# Autodesk Inventor assembly: mg996r 3mm center frame
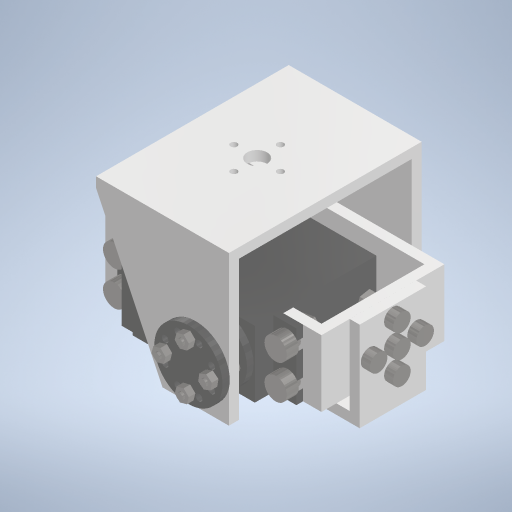
[picture p0: Inventor's stored thumbnail of the model, 512x512]
Saved by Autodesk Inventor 2023 (Build 270158000, 158)
## iProperties
Created: 2022-06-29
Part Number: mg996r 3mm center frame
Document SubType Name: Assembly
Designer: isamu
Author: isamu
## iProperties of the stored document servo frame mg996 centered.ipt
Created: 2022-06-29
Part Number: Pocket036
Material: Generic
Description: FreeCAD Model
Document SubType Name: Modeling
Designer: isamu
Authority: Unknown
Density: 1 g/cm^3
Appearance: Default
Title: Open CASCADE Shape Model
Author: Author
Sending System: FreeCAD
Preprocessor: Open CASCADE STEP processor 7.5
## Documents named in this file (7)
- **D:\personal_projects\robot\inventor\mg996r 3mm center frame.iam*LocalDocs*xAaaaawdaAaaaaaaaAaaaajx33d*servo frame mg996 centered.ipt
- D:\personal_projects\robot\inventor\mg996r 3mm center frame.iam
- D:\personal_projects\robot\inventor\base mg996r 3mm with bottom.iam
- D:\personal_projects\robot\exports\frames\m4 nuts.ipt
- D:\personal_projects\robot\exports\frames\m2x8.ipt
- D:\personal_projects\robot\exports\frames\m2 nuts.ipt
- D:\personal_projects\robot\exports\frames\servo frame mg996 centered.step
## Components (11 placed, 5 different names)
1. base mg996r 3mm with bottom:1 [sub-assembly] — Insert:6, Insert:7, Insert:8, Insert:9, Mate:1, Mate:2, Mate:3
2. m4 nuts:1 — Insert:10
3. m2x8:1 — Insert:12
4. m2x8:2 — Insert:13
5. m2x8:3 — Insert:11
6. m2x8:4 — Insert:14
7. m2 nuts:1 — Insert:6
8. m2 nuts:2 — Insert:9
9. m2 nuts:3 — Insert:8
10. m2 nuts:4 — Insert:7
11. servo frame mg996 centered:1 — Mate:1, Mate:2, Mate:3, Insert:10, Insert:11, Insert:12, Insert:13, Insert:14
## Relationships (12: Insert 9, Mate 3)
- Insert:6: base mg996r 3mm with bottom:1 ↔ m2 nuts:1
- Insert:7: base mg996r 3mm with bottom:1 ↔ m2 nuts:4
- Insert:8: base mg996r 3mm with bottom:1 ↔ m2 nuts:3
- Insert:9: base mg996r 3mm with bottom:1 ↔ m2 nuts:2
- Mate:1: base mg996r 3mm with bottom:1 ↔ servo frame mg996 centered:1
- Mate:2: base mg996r 3mm with bottom:1 ↔ servo frame mg996 centered:1
- Mate:3: base mg996r 3mm with bottom:1 ↔ servo frame mg996 centered:1
- Insert:10: m4 nuts:1 ↔ servo frame mg996 centered:1
- Insert:11: m2x8:3 ↔ servo frame mg996 centered:1
- Insert:12: m2x8:1 ↔ servo frame mg996 centered:1
- Insert:13: m2x8:2 ↔ servo frame mg996 centered:1
- Insert:14: m2x8:4 ↔ servo frame mg996 centered:1
